# Autodesk Inventor assembly: WireBarrelComponent
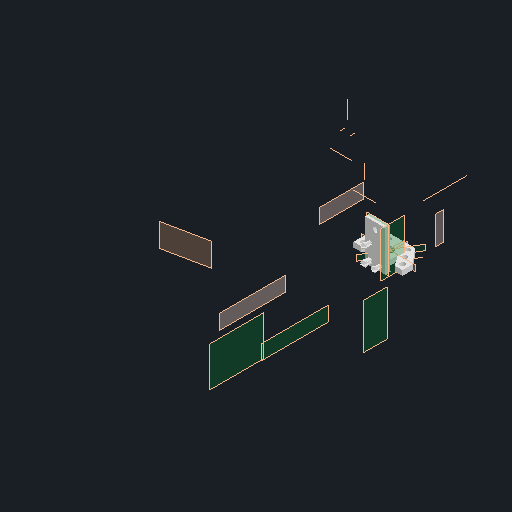
[picture p0: Inventor's stored thumbnail of the model, 512x512]
Saved by Autodesk Inventor 2024.1 (Build 281209000, 209)
## iProperties
Created: 2023-08-17
Part Number: WireBarrelComponent
Document SubType Name: Assembly
Designer: Eleanor
Author: Eleanor
## Documents named in this file (3)
- C:\Users\Eleanor\Documents\Inventor\4.5mm ERS\WireBarrelComponent.iam
- C:\Users\Eleanor\Documents\Inventor\4.5mm ERS\WireSlottedHoles.iam
- C:\Users\Eleanor\Documents\Inventor\4.5mm ERS\MirrorBaseplate_MIR.ipt
## Components (2 placed, 2 different names)
1. WireSlottedHoles:1 [sub-assembly] — Mate:16, Mate:17, Angle:4, Mate:21, Mate:25, Mate:28, Mate:32, Mate:34
2. MirrorBaseplate_MIR:1 — Mate:32, Mate:33, Angle:5, Symmetry:1
## Relationships (14: Mate 11, Angle 2, Symmetry 1)
- Mate:7
- Mate:14
- Mate:16: WireSlottedHoles:1
- Mate:17: WireSlottedHoles:1
- Mate:20
- Angle:4 (90 deg): WireSlottedHoles:1
- Mate:21: WireSlottedHoles:1
- Mate:25: WireSlottedHoles:1
- Mate:28: WireSlottedHoles:1
- Mate:32: WireSlottedHoles:1 ↔ MirrorBaseplate_MIR:1
- Mate:33: MirrorBaseplate_MIR:1
- Angle:5 (0 deg): MirrorBaseplate_MIR:1
- Symmetry:1: MirrorBaseplate_MIR:1
- Mate:34: WireSlottedHoles:1
